# Autodesk Inventor assembly: capsule.top.assembly
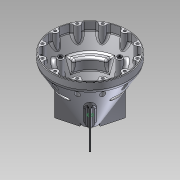
[picture p0: Inventor's stored thumbnail of the model, 180x180]
Saved by Autodesk Inventor 2011 (Build 150239000, 239)
## iProperties
Created: 2011-01-27
Part Number: capsule.top.assembly
Document SubType Name: Assembly
Designer: Casey
Author: Casey
## Documents named in this file (5)
- C:\Users\Rob\Dropbox\RockSAT-X 2011 RexSAT\capsule-launcher.design\Capsule\capsule.top.assembly.iam
- C:\Users\Rob\Dropbox\RockSAT-X 2011 RexSAT\capsule-launcher.design\Capsule\Capsule.top.ipt
- C:\Users\Rob\Dropbox\RockSAT-X 2011 RexSAT\capsule-launcher.design\Capsule\capsule.fin.ipt
- C:\Users\Rob\Dropbox\RockSAT-X 2011 RexSAT\capsule-launcher.design\ANSI B18.3.1M(6)\ANSI B18.3.1M - M3x0.5 x 12(1).ipt
- C:\Users\Rob\Dropbox\RockSAT-X 2011 RexSAT\capsule-launcher.design\Capsule\Capsule.contactring.ipt
## Components (11 placed, 4 different names)
1. Capsule.top:1 — Tangent:2, Insert:11, Mate:1, Mate:2, Mate:3, Tangent:3, Tangent:4, Mate:4, Mate:5, Mate:6
2. capsule.fin:1 — Tangent:2, Mate:1, Mate:4
3. capsule.fin:2 — Mate:3, Tangent:3, Mate:6
4. capsule.fin:3 — Mate:2, Tangent:4, Mate:5
5. Forged Socket Head Cap Screw - Metric M3x0.5 x 12:1
6. Forged Socket Head Cap Screw - Metric M3x0.5 x 12:2
7. Forged Socket Head Cap Screw - Metric M3x0.5 x 12:3
8. Forged Socket Head Cap Screw - Metric M3x0.5 x 12:4
9. Forged Socket Head Cap Screw - Metric M3x0.5 x 12:5
10. Forged Socket Head Cap Screw - Metric M3x0.5 x 12:6
11. Capsule.contactring:1 — Insert:11
## Relationships (10: Mate 6, Tangent 3, Insert 1)
- Tangent:2: Capsule.top:1 ↔ capsule.fin:1
- Insert:11: Capsule.top:1 ↔ Capsule.contactring:1
- Mate:1: Capsule.top:1 ↔ capsule.fin:1
- Mate:2: Capsule.top:1 ↔ capsule.fin:3
- Mate:3: Capsule.top:1 ↔ capsule.fin:2
- Tangent:3: Capsule.top:1 ↔ capsule.fin:2
- Tangent:4: Capsule.top:1 ↔ capsule.fin:3
- Mate:4: Capsule.top:1 ↔ capsule.fin:1
- Mate:5: Capsule.top:1 ↔ capsule.fin:3
- Mate:6: Capsule.top:1 ↔ capsule.fin:2
